# Autodesk Inventor assembly: On-Off Switch
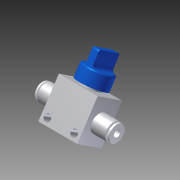
[picture p0: Inventor's stored thumbnail of the model, 180x180]
Saved by Autodesk Inventor 2012 (Build 160160000, 160)
## iProperties
Created: 2011-03-21
Part Number: On-Off Switch
Document SubType Name: Assembly
Designer: Jordan
Translation Standard: STEP AP203
FileName: VHVHK3-1203418587055.step
PreProcessor: SolidWorks 2009
PostProcessor: Build: 239, Release: 2011 RTM - Date: Wed 02/17/2010
Sent Units: millimeter
Uncertainty: 1e-05
Author: Jordan
## Documents named in this file (4)
- C:\Users\Wade\Documents\24C VEX CAD Files\Other Parts\On-Off Switch.iam
- C:\Users\Wade\Documents\24C VEX CAD Files\Other Parts\On-Off Switch-Parts\Fitting.ipt
- C:\Users\Wade\Documents\24C VEX CAD Files\Other Parts\On-Off Switch-Parts\Knob.ipt
- C:\Users\Wade\Documents\24C VEX CAD Files\Other Parts\On-Off Switch-Parts\On-Off Switch Body.ipt
## Components (4 placed, 3 different names)
1. Fitting:1 — Mate:2, Flush:1
2. Knob:1 — Mate:3, Mate:4, Angle:1
3. Fitting:2 — Mate:1, Flush:2
4. On-Off Switch Body:1 — Mate:1, Mate:2, Flush:1, Flush:2, Mate:3, Mate:4, Angle:1
## Relationships (7: Mate 4, Flush 2, Angle 1)
- Mate:1: Fitting:2 ↔ On-Off Switch Body:1
- Mate:2: Fitting:1 ↔ On-Off Switch Body:1
- Flush:1: Fitting:1 ↔ On-Off Switch Body:1
- Flush:2: Fitting:2 ↔ On-Off Switch Body:1
- Mate:3: Knob:1 ↔ On-Off Switch Body:1
- Mate:4: Knob:1 ↔ On-Off Switch Body:1
- Angle:1 (0 deg): Knob:1 ↔ On-Off Switch Body:1
